# Autodesk Inventor assembly: Top_Backboard Assy
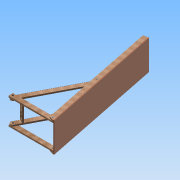
[picture p0: Inventor's stored thumbnail of the model, 180x180]
Saved by Autodesk Inventor 2018.1 (Build 221171000, 171)
## iProperties
Created: 2019-03-15
Part Number: Top_Backboard Assy
Document SubType Name: Assembly
Designer: James
Author: James
## Documents named in this file (15)
- C:\Users\admin\Desktop\Ball-Machine\Top Level\Top_Backboard Assy.iam
- C:\Users\admin\Desktop\Ball-Machine\Top Level\Top_Backboard.ipt
- C:\Users\admin\Desktop\Ball-Machine\Top Level\Top_Reinforcement 2.ipt
- C:\Users\admin\Desktop\Ball-Machine\Top Level\Top_Reinforcement_LHS.ipt
- C:\Users\admin\Desktop\Ball-Machine\Top Level\Top_Reinforcement_RHS.ipt
- C:\Users\admin\Desktop\Ball-Machine\Top Level\Din97 - 8x80 - Steel Wood Screw.ipt
- C:\Users\admin\Desktop\Ball-Machine\Top Level\Top_Hinge Cylinder.ipt
- C:\Users\admin\Desktop\Ball-Machine\Top Level\Top_Hinge End.ipt
- C:\Users\admin\Desktop\Ball-Machine\Top Level\Socket Cap Screw - Standard - (A2) - M8 x 20.ipt
- C:\Users\admin\Desktop\Ball-Machine\Top Level\Top_Floor Plank.ipt
- C:\Users\admin\Desktop\Ball-Machine\Top Level\Top_Reinforcement 3.ipt
- C:\Users\admin\Desktop\Ball-Machine\Top Level\Top_Rear Plank_RHS.ipt
- C:\Users\admin\Desktop\Ball-Machine\Top Level\Top_Rear Plank_LHS.ipt
- C:\Users\admin\Desktop\Ball-Machine\Top Level\Top_Spacer.ipt
- C:\Users\admin\Desktop\Ball-Machine\Top Level\Top_Hinge Cylinder Long.ipt
## Components (55 placed, 14 different names)
1. Top_Backboard:1 — Flush:3, Mate:1, Mate:2, Flush:5, Flush:6, Flush:7, Flush:8, Flush:10, Mate:5
2. Top_Reinforcement_LHS:1 — Mate:1, Flush:4, Flush:5, Flush:6, Flush:10, Mate:3, Mate:6, Mate:7, Mate:12, Mate:13, Flush:12, Mate:14, Mate:15, Mate:20, Mate:23, Mate:32, Mate:73, Mate:74, Mate:75, Mate:76, Mate:77, Mate:89, Mate:90
3. Top_Reinforcement_RHS:1 — Mate:2, Flush:4, Flush:7, Flush:8, Mate:4, Mate:8, Mate:9, Mate:10, Mate:11, Flush:13, Mate:21, Mate:22, Mate:31, Mate:55, Mate:56, Mate:64, Mate:65, Mate:66, Mate:67, Mate:68, Mate:82, Mate:83
4. Top_Floor Plank:1 — Mate:21, Mate:22, Flush:15, Mate:29, Mate:30, Mate:57, Mate:58, Mate:59
5. Top_Floor Plank:2 — Mate:20, Mate:23, Flush:15, Mate:24, Mate:25, Mate:26, Mate:27, Mate:28, Mate:61, Mate:62
6. Top_Rear Plank_RHS:1 — Mate:29, Mate:30, Flush:16, Mate:31, Mate:36, Mate:37, Mate:38, Mate:41, Mate:42, Flush:17, Mate:60, Mate:84, Mate:85
7. Top_Rear Plank_LHS:1 — Mate:27, Mate:28, Flush:16, Mate:32, Mate:33, Mate:34, Mate:35, Mate:39, Mate:40, Flush:20, Mate:63, Mate:91
8. Top_Reinforcement 3:1 — Mate:33, Mate:34, Mate:35, Mate:36, Mate:37, Mate:38
9. Top_Spacer:1 — Mate:64, Mate:65, Mate:66, Mate:67, Mate:68, Mate:69, Mate:70, Mate:71, Mate:72, Flush:24
10. Top_Spacer:2 — Mate:73, Mate:74, Mate:75, Mate:76, Mate:77, Flush:28, Mate:78, Mate:79, Mate:80, Mate:81
11. Top_Hinge End:6 — Mate:91, Mate:92, Mate:93, Mate:94, Mate:95
12. Top_Hinge Cylinder Long:2 — Mate:89, Mate:90, Mate:92, Mate:93
13. Din97 - 8x80 - Steel Wood Screw:17 — Mate:69, Flush:21
14. Din97 - 8x80 - Steel Wood Screw:18 — Mate:70, Flush:21, Flush:22, Flush:23, Flush:24
15. Din97 - 8x80 - Steel Wood Screw:19 — Mate:71, Flush:23
16. Din97 - 8x80 - Steel Wood Screw:20 — Mate:72, Flush:22
17. Din97 - 8x80 - Steel Wood Screw:21 — Flush:25, Flush:26, Flush:27, Flush:28, Mate:78
18. Din97 - 8x80 - Steel Wood Screw:22 — Flush:25, Mate:79
19. Din97 - 8x80 - Steel Wood Screw:23 — Flush:26, Mate:80
20. Din97 - 8x80 - Steel Wood Screw:24 — Flush:27, Mate:81
21. Socket Cap Screw - Standard - (A2) - M8 x 20:5 — Mate:87, Mate:88
22. Top_Hinge Cylinder Long:1 — Mate:82, Mate:83, Mate:86
23. Top_Hinge End:5 — Mate:84, Mate:85, Mate:86, Mate:87, Mate:88
24. Socket Cap Screw - Standard - (A2) - M8 x 20:6 — Mate:94, Mate:95
25. Socket Cap Screw - Standard - (A2) - M8 x 20:4
26. Top_Hinge End:4 — Mate:57
27. Top_Hinge Cylinder:4 — Mate:55, Mate:56
28. Socket Cap Screw - Standard - (A2) - M8 x 20:3
29. Top_Hinge End:3 — Mate:60
30. Top_Hinge Cylinder:3 — Mate:58, Mate:59
31. Socket Cap Screw - Standard - (A2) - M8 x 20:2
32. Top_Hinge End:2 — Mate:63
33. Top_Hinge Cylinder:2 — Mate:61, Mate:62
34. Din97 - 8x80 - Steel Wood Screw:16 — Mate:41, Flush:18
35. Din97 - 8x80 - Steel Wood Screw:15 — Mate:42, Flush:17, Flush:18
36. Din97 - 8x80 - Steel Wood Screw:14 — Mate:40, Flush:19, Flush:20
37. Din97 - 8x80 - Steel Wood Screw:13 — Mate:39, Flush:19
38. Socket Cap Screw - Standard - (A2) - M8 x 20:1 — Mate:18, Mate:19
39. Top_Hinge End:1 — Mate:16, Mate:17, Mate:18, Mate:19, Mate:26
40. Top_Hinge Cylinder:1 — Mate:14, Mate:15, Mate:16, Mate:17
41. Top_Reinforcement 2:1 — Mate:3, Mate:4, Mate:5, Mate:6, Mate:7, Mate:8, Mate:9
42. Din97 - 8x80 - Steel Wood Screw:1 — Mate:10, Flush:13, Flush:14
43. Din97 - 8x80 - Steel Wood Screw:2 — Mate:11, Flush:14
44. Din97 - 8x80 - Steel Wood Screw:3 — Mate:12, Flush:11, Flush:12
45. Din97 - 8x80 - Steel Wood Screw:4 — Mate:13, Flush:11
46. Top_Reinforcement 2:2
47. Din97 - 8x80 - Steel Wood Screw:5
48. Din97 - 8x80 - Steel Wood Screw:6
49. Din97 - 8x80 - Steel Wood Screw:7
50. Din97 - 8x80 - Steel Wood Screw:8
51. Top_Reinforcement 2:3
52. Din97 - 8x80 - Steel Wood Screw:9
53. Din97 - 8x80 - Steel Wood Screw:10
54. Din97 - 8x80 - Steel Wood Screw:11
55. Din97 - 8x80 - Steel Wood Screw:12
## Component patterns: (3 elements, first: Top_Reinforcement 2:1 + Din97 - 8x80 - Steel Wood Screw:1 + Din97 - 8x80 - Steel Wood Screw:2 + Din97 - 8x80 - Steel Wood Screw:3 + Din97 - 8x80 - Steel Wood Screw:4)
## Relationships (120: Mate 95, Flush 25)
- Flush:3: Top_Backboard:1
- Mate:1: Top_Backboard:1 ↔ Top_Reinforcement_LHS:1
- Mate:2: Top_Backboard:1 ↔ Top_Reinforcement_RHS:1
- Flush:4: Top_Reinforcement_LHS:1 ↔ Top_Reinforcement_RHS:1
- Flush:5: Top_Backboard:1 ↔ Top_Reinforcement_LHS:1
- Flush:6: Top_Backboard:1 ↔ Top_Reinforcement_LHS:1
- Flush:7: Top_Backboard:1 ↔ Top_Reinforcement_RHS:1
- Flush:8: Top_Backboard:1 ↔ Top_Reinforcement_RHS:1
- Flush:10: Top_Backboard:1 ↔ Top_Reinforcement_LHS:1
- Mate:3: Top_Reinforcement_LHS:1 ↔ Top_Reinforcement 2:1
- Mate:4: Top_Reinforcement_RHS:1 ↔ Top_Reinforcement 2:1
- Mate:5: Top_Backboard:1 ↔ Top_Reinforcement 2:1
- Mate:6: Top_Reinforcement_LHS:1 ↔ Top_Reinforcement 2:1
- Mate:7: Top_Reinforcement_LHS:1 ↔ Top_Reinforcement 2:1
- Mate:8: Top_Reinforcement_RHS:1 ↔ Top_Reinforcement 2:1
- Mate:9: Top_Reinforcement_RHS:1 ↔ Top_Reinforcement 2:1
- Mate:10: Top_Reinforcement_RHS:1 ↔ Din97 - 8x80 - Steel Wood Screw:1
- Mate:11: Top_Reinforcement_RHS:1 ↔ Din97 - 8x80 - Steel Wood Screw:2
- Mate:12: Top_Reinforcement_LHS:1 ↔ Din97 - 8x80 - Steel Wood Screw:3
- Mate:13: Top_Reinforcement_LHS:1 ↔ Din97 - 8x80 - Steel Wood Screw:4
- Flush:11: Din97 - 8x80 - Steel Wood Screw:3 ↔ Din97 - 8x80 - Steel Wood Screw:4
- Flush:12: Top_Reinforcement_LHS:1 ↔ Din97 - 8x80 - Steel Wood Screw:3
- Flush:13: Top_Reinforcement_RHS:1 ↔ Din97 - 8x80 - Steel Wood Screw:1
- Flush:14: Din97 - 8x80 - Steel Wood Screw:1 ↔ Din97 - 8x80 - Steel Wood Screw:2
- Mate:14: Top_Reinforcement_LHS:1 ↔ Top_Hinge Cylinder:1
- Mate:15: Top_Reinforcement_LHS:1 ↔ Top_Hinge Cylinder:1
- Mate:16: Top_Hinge End:1 ↔ Top_Hinge Cylinder:1
- Mate:17: Top_Hinge End:1 ↔ Top_Hinge Cylinder:1
- Mate:18: Socket Cap Screw - Standard - (A2) - M8 x 20:1 ↔ Top_Hinge End:1
- Mate:19: Socket Cap Screw - Standard - (A2) - M8 x 20:1 ↔ Top_Hinge End:1
- Mate:20: Top_Reinforcement_LHS:1 ↔ Top_Floor Plank:2
- Mate:21: Top_Reinforcement_RHS:1 ↔ Top_Floor Plank:1
- Mate:22: Top_Reinforcement_RHS:1 ↔ Top_Floor Plank:1
- Mate:23: Top_Reinforcement_LHS:1 ↔ Top_Floor Plank:2
- Flush:15: Top_Floor Plank:1 ↔ Top_Floor Plank:2
- Mate:24: Top_Floor Plank:2
- Mate:25: Top_Floor Plank:2
- Mate:26: Top_Floor Plank:2 ↔ Top_Hinge End:1
- Mate:27: Top_Floor Plank:2 ↔ Top_Rear Plank_LHS:1
- Mate:28: Top_Floor Plank:2 ↔ Top_Rear Plank_LHS:1
- Mate:29: Top_Floor Plank:1 ↔ Top_Rear Plank_RHS:1
- Mate:30: Top_Floor Plank:1 ↔ Top_Rear Plank_RHS:1
- Flush:16: Top_Rear Plank_RHS:1 ↔ Top_Rear Plank_LHS:1
- Mate:31: Top_Reinforcement_RHS:1 ↔ Top_Rear Plank_RHS:1
- Mate:32: Top_Reinforcement_LHS:1 ↔ Top_Rear Plank_LHS:1
- Mate:33: Top_Rear Plank_LHS:1 ↔ Top_Reinforcement 3:1
- Mate:34: Top_Rear Plank_LHS:1 ↔ Top_Reinforcement 3:1
- Mate:35: Top_Rear Plank_LHS:1 ↔ Top_Reinforcement 3:1
- Mate:36: Top_Rear Plank_RHS:1 ↔ Top_Reinforcement 3:1
- Mate:37: Top_Rear Plank_RHS:1 ↔ Top_Reinforcement 3:1
- Mate:38: Top_Rear Plank_RHS:1 ↔ Top_Reinforcement 3:1
- Mate:39: Top_Rear Plank_LHS:1 ↔ Din97 - 8x80 - Steel Wood Screw:13
- Mate:40: Top_Rear Plank_LHS:1 ↔ Din97 - 8x80 - Steel Wood Screw:14
- Mate:41: Top_Rear Plank_RHS:1 ↔ Din97 - 8x80 - Steel Wood Screw:16
- Mate:42: Top_Rear Plank_RHS:1 ↔ Din97 - 8x80 - Steel Wood Screw:15
- Flush:17: Top_Rear Plank_RHS:1 ↔ Din97 - 8x80 - Steel Wood Screw:15
- Flush:18: Din97 - 8x80 - Steel Wood Screw:16 ↔ Din97 - 8x80 - Steel Wood Screw:15
- Flush:19: Din97 - 8x80 - Steel Wood Screw:14 ↔ Din97 - 8x80 - Steel Wood Screw:13
- Flush:20: Top_Rear Plank_LHS:1 ↔ Din97 - 8x80 - Steel Wood Screw:14
- [Mate]: Top_Hinge End:2 ↔ Top_Hinge Cylinder:2
- [Mate]: Top_Hinge End:2 ↔ Top_Hinge Cylinder:2
- [Mate]: Socket Cap Screw - Standard - (A2) - M8 x 20:2 ↔ Top_Hinge End:2
- [Mate]: Socket Cap Screw - Standard - (A2) - M8 x 20:2 ↔ Top_Hinge End:2
- [Mate]: Top_Hinge End:3 ↔ Top_Hinge Cylinder:3
- [Mate]: Top_Hinge End:3 ↔ Top_Hinge Cylinder:3
- [Mate]: Socket Cap Screw - Standard - (A2) - M8 x 20:3 ↔ Top_Hinge End:3
- [Mate]: Socket Cap Screw - Standard - (A2) - M8 x 20:3 ↔ Top_Hinge End:3
- [Mate]: Top_Hinge End:4 ↔ Top_Hinge Cylinder:4
- [Mate]: Top_Hinge End:4 ↔ Top_Hinge Cylinder:4
- [Mate]: Socket Cap Screw - Standard - (A2) - M8 x 20:4 ↔ Top_Hinge End:4
- [Mate]: Socket Cap Screw - Standard - (A2) - M8 x 20:4 ↔ Top_Hinge End:4
- Mate:55: Top_Reinforcement_RHS:1 ↔ Top_Hinge Cylinder:4
- Mate:56: Top_Reinforcement_RHS:1 ↔ Top_Hinge Cylinder:4
- Mate:57: Top_Floor Plank:1 ↔ Top_Hinge End:4
- Mate:58: Top_Floor Plank:1 ↔ Top_Hinge Cylinder:3
- Mate:59: Top_Floor Plank:1 ↔ Top_Hinge Cylinder:3
- Mate:60: Top_Rear Plank_RHS:1 ↔ Top_Hinge End:3
- Mate:61: Top_Floor Plank:2 ↔ Top_Hinge Cylinder:2
- Mate:62: Top_Floor Plank:2 ↔ Top_Hinge Cylinder:2
- Mate:63: Top_Rear Plank_LHS:1 ↔ Top_Hinge End:2
- Mate:64: Top_Reinforcement_RHS:1 ↔ Top_Spacer:1
- Mate:65: Top_Reinforcement_RHS:1 ↔ Top_Spacer:1
- Mate:66: Top_Reinforcement_RHS:1 ↔ Top_Spacer:1
- Mate:67: Top_Reinforcement_RHS:1 ↔ Top_Spacer:1
- Mate:68: Top_Reinforcement_RHS:1 ↔ Top_Spacer:1
- Mate:69: Top_Spacer:1 ↔ Din97 - 8x80 - Steel Wood Screw:17
- Mate:70: Top_Spacer:1 ↔ Din97 - 8x80 - Steel Wood Screw:18
- Mate:71: Top_Spacer:1 ↔ Din97 - 8x80 - Steel Wood Screw:19
- Mate:72: Top_Spacer:1 ↔ Din97 - 8x80 - Steel Wood Screw:20
- Flush:21: Din97 - 8x80 - Steel Wood Screw:17 ↔ Din97 - 8x80 - Steel Wood Screw:18
- Flush:22: Din97 - 8x80 - Steel Wood Screw:18 ↔ Din97 - 8x80 - Steel Wood Screw:20
- Flush:23: Din97 - 8x80 - Steel Wood Screw:18 ↔ Din97 - 8x80 - Steel Wood Screw:19
- Flush:24: Top_Spacer:1 ↔ Din97 - 8x80 - Steel Wood Screw:18
- Mate:73: Top_Reinforcement_LHS:1 ↔ Top_Spacer:2
- Mate:74: Top_Reinforcement_LHS:1 ↔ Top_Spacer:2
- Mate:75: Top_Reinforcement_LHS:1 ↔ Top_Spacer:2
- Mate:76: Top_Reinforcement_LHS:1 ↔ Top_Spacer:2
- Mate:77: Top_Reinforcement_LHS:1 ↔ Top_Spacer:2
- Flush:25: Din97 - 8x80 - Steel Wood Screw:21 ↔ Din97 - 8x80 - Steel Wood Screw:22
- Flush:26: Din97 - 8x80 - Steel Wood Screw:21 ↔ Din97 - 8x80 - Steel Wood Screw:23
- Flush:27: Din97 - 8x80 - Steel Wood Screw:21 ↔ Din97 - 8x80 - Steel Wood Screw:24
- Flush:28: Top_Spacer:2 ↔ Din97 - 8x80 - Steel Wood Screw:21
- Mate:78: Top_Spacer:2 ↔ Din97 - 8x80 - Steel Wood Screw:21
- Mate:79: Top_Spacer:2 ↔ Din97 - 8x80 - Steel Wood Screw:22
- Mate:80: Top_Spacer:2 ↔ Din97 - 8x80 - Steel Wood Screw:23
- Mate:81: Top_Spacer:2 ↔ Din97 - 8x80 - Steel Wood Screw:24
- Mate:82: Top_Reinforcement_RHS:1 ↔ Top_Hinge Cylinder Long:1
- Mate:83: Top_Reinforcement_RHS:1 ↔ Top_Hinge Cylinder Long:1
- Mate:84: Top_Rear Plank_RHS:1 ↔ Top_Hinge End:5
- Mate:85: Top_Rear Plank_RHS:1 ↔ Top_Hinge End:5
- Mate:86: Top_Hinge Cylinder Long:1 ↔ Top_Hinge End:5
- Mate:87: Socket Cap Screw - Standard - (A2) - M8 x 20:5 ↔ Top_Hinge End:5
- Mate:88: Socket Cap Screw - Standard - (A2) - M8 x 20:5 ↔ Top_Hinge End:5
- Mate:89: Top_Reinforcement_LHS:1 ↔ Top_Hinge Cylinder Long:2
- Mate:90: Top_Reinforcement_LHS:1 ↔ Top_Hinge Cylinder Long:2
- Mate:91: Top_Rear Plank_LHS:1 ↔ Top_Hinge End:6
- Mate:92: Top_Hinge End:6 ↔ Top_Hinge Cylinder Long:2
- Mate:93: Top_Hinge End:6 ↔ Top_Hinge Cylinder Long:2
- Mate:94: Top_Hinge End:6 ↔ Socket Cap Screw - Standard - (A2) - M8 x 20:6
- Mate:95: Top_Hinge End:6 ↔ Socket Cap Screw - Standard - (A2) - M8 x 20:6
## Named parameters: d66_d33 = 0 mm, d67_d34 = 0 mm, d68_d35 = 0 mm, d69_d36 = 0 mm, d70_d33 = 0 mm, d71_d34 = 0 mm, d72_d35 = 0 mm, d73_d36 = 0 mm, d74_d33 = 0 mm, d75_d34 = 0 mm, d76_d35 = 0 mm, d77_d36 = 0 mm
